# Autodesk Inventor assembly: aRM V3
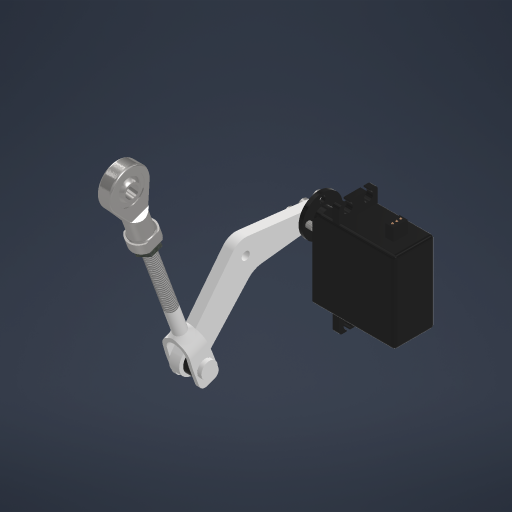
[picture p0: Inventor's stored thumbnail of the model, 512x512]
Saved by Autodesk Inventor 2023 (Build 270158000, 158)
## iProperties
Created: 2023-03-12
Part Number: aRM V3
Document SubType Name: Assembly
Designer: roota
Author: roota
## Documents named in this file (10)
- D:\GitHub\NTUST-Mechanical-Design\Ball stabilization mechanism\3D CAD files\Mechanical Part CAD files\Assemblies\Arm v3.iam
- D:\GitHub\NTUST-Mechanical-Design\Ball stabilization mechanism\3D CAD files\Electrical Hardware CAD files\SERVO\LDX-335MG_Servo_15kg_cm.ipt
- D:\GitHub\NTUST-Mechanical-Design\Ball stabilization mechanism\3D CAD files\Electrical Hardware CAD files\SERVO\ServoDrive.ipt
- D:\GitHub\NTUST-Mechanical-Design\Ball stabilization mechanism\3D CAD files\Mechanical Part CAD files\Hardware Parts\LKBK4-L43-S41-Q130-M3-HA6-T5.ipt
- D:\GitHub\NTUST-Mechanical-Design\Ball stabilization mechanism\3D CAD files\Mechanical Part CAD files\Hardware Parts\M6x1 Welded thread fork\M6x1 Welded thread fork.ipt
- D:\GitHub\NTUST-Mechanical-Design\Ball stabilization mechanism\3D CAD files\Mechanical Part CAD files\Static Mechanisms\4mm spacer.ipt
- D:\GitHub\NTUST-Mechanical-Design\Ball stabilization mechanism\3D CAD files\Mechanical Part CAD files\Hardware Parts\SELF-LUBRIFICATING ROD END\End_6mm.ipt
- D:\GitHub\NTUST-Mechanical-Design\Ball stabilization mechanism\3D CAD files\Mechanical Part CAD files\Hardware Parts\SELF-LUBRIFICATING ROD END\Ball_6mm_male.ipt
- C:\Users\roota\Documents\Inventor\Content Center Files\R2023\en-US\ISO 4036(2)\ISO 4036 - M6(2).ipt
- C:\Users\roota\Documents\Inventor\Content Center Files\R2023\en-US\ISO 4762(2)\ISO 4762 - M3 x 10ISO.ipt
## Components (11 placed, 9 different names)
1. LDX-335MG_Servo_15kg_cm:1 — Mate:1, Mate:2, Mate:3, Insert:1
2. ServoDrive:1 — Insert:1, Insert:2, Mate:4
3. LKBK4-L43-S41-Q130-M3-HA6-T5:1 — Insert:2, Mate:4, Insert:3, Angle:1, Insert:7, Insert:8, Insert:9
4. M6x1 Welded thread fork:1 — Insert:3, Insert:4, Insert:5
5. 4mm spacer:1 — Insert:4
6. End_6mm:1 — Insert:5, Angle:1, Tangent:1, Insert:6
7. Ball_6mm_male:1 — Tangent:1
8. ISO 4036 M6:1 — Insert:6
9. ISO 4762 M3 x 10:1 — Insert:7
10. ISO 4762 M3 x 10:2 — Insert:8
11. ISO 4762 M3 x 10:3 — Insert:9
## Relationships (15: Insert 9, Mate 4, Angle 1, Tangent 1)
- Mate:1: LDX-335MG_Servo_15kg_cm:1
- Mate:2: LDX-335MG_Servo_15kg_cm:1
- Mate:3: LDX-335MG_Servo_15kg_cm:1
- Insert:1: LDX-335MG_Servo_15kg_cm:1 ↔ ServoDrive:1
- Insert:2: ServoDrive:1 ↔ LKBK4-L43-S41-Q130-M3-HA6-T5:1
- Mate:4: ServoDrive:1 ↔ LKBK4-L43-S41-Q130-M3-HA6-T5:1
- Insert:3: LKBK4-L43-S41-Q130-M3-HA6-T5:1 ↔ M6x1 Welded thread fork:1
- Insert:4: M6x1 Welded thread fork:1 ↔ 4mm spacer:1
- Insert:5 (-10 mm): M6x1 Welded thread fork:1 ↔ End_6mm:1
- Angle:1 (0 deg): LKBK4-L43-S41-Q130-M3-HA6-T5:1 ↔ End_6mm:1
- Tangent:1: End_6mm:1 ↔ Ball_6mm_male:1
- Insert:6: End_6mm:1 ↔ ISO 4036 M6:1
- Insert:7: LKBK4-L43-S41-Q130-M3-HA6-T5:1 ↔ ISO 4762 M3 x 10:1
- Insert:8: LKBK4-L43-S41-Q130-M3-HA6-T5:1 ↔ ISO 4762 M3 x 10:2
- Insert:9: LKBK4-L43-S41-Q130-M3-HA6-T5:1 ↔ ISO 4762 M3 x 10:3
